# Autodesk Inventor assembly: SailAssembly
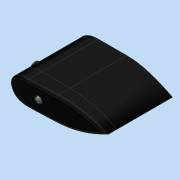
[picture p0: Inventor's stored thumbnail of the model, 180x180]
Saved by Autodesk Inventor 2017.3 (Build 213256000, 256)
## iProperties
Created: 2018-02-22
Part Number: SailAssembly
Document SubType Name: Assembly
Designer: Derek Wider
Author: Derek Wider
## Documents named in this file (6)
- G:\Projects\Submarine\Submarine-project\CAD\midships\Sail\SailAssembly\SailAssembly.iam
- G:\Projects\Submarine\Submarine-project\CAD\midships\Sail\SailAssembly\SailBottom.ipt
- G:\Projects\Submarine\Submarine-project\CAD\midships\Sail\SailAssembly\SailTop.ipt
- G:\Projects\Submarine\Submarine-project\CAD\midships\Sail\camera\CameraAssembly.iam
- G:\Projects\Submarine\Submarine-project\CAD\common\screws\flatPlasticScrewSmall.ipt
- G:\Projects\Submarine\Submarine-project\CAD\common\5mmLED.ipt
## Components (6 placed, 5 different names)
1. SailBottom:1 — Mate:1, Angle:1, Tangent:1, Mate:2, Flush:1, Mate:3, Flush:2, Flush:3, Mate:7
2. SailTop:1 — Mate:2, Flush:1, Mate:3, Mate:4, Mate:5, Mate:6
3. CameraAssembly:1 [sub-assembly] — Mate:1, Angle:1, Tangent:1
4. flatPlasticScrewSmall:1 — Mate:4, Flush:3
5. flatPlasticScrewSmall:2 — Mate:5, Flush:2
6. 5mmLED:1 — Mate:6, Mate:7
## Relationships (12: Mate 7, Flush 3, Angle 1, Tangent 1)
- Mate:1: SailBottom:1 ↔ CameraAssembly:1
- Angle:1 (0 deg): SailBottom:1 ↔ CameraAssembly:1
- Tangent:1: SailBottom:1 ↔ CameraAssembly:1
- Mate:2: SailBottom:1 ↔ SailTop:1
- Flush:1: SailBottom:1 ↔ SailTop:1
- Mate:3: SailBottom:1 ↔ SailTop:1
- Mate:4: SailTop:1 ↔ flatPlasticScrewSmall:1
- Mate:5: SailTop:1 ↔ flatPlasticScrewSmall:2
- Flush:2: SailBottom:1 ↔ flatPlasticScrewSmall:2
- Flush:3: SailBottom:1 ↔ flatPlasticScrewSmall:1
- Mate:6: SailTop:1 ↔ 5mmLED:1
- Mate:7 (6.35 mm): SailBottom:1 ↔ 5mmLED:1
